# Autodesk Inventor assembly: base_roulante_pmi
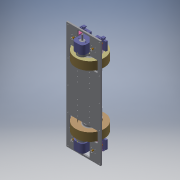
[picture p0: Inventor's stored thumbnail of the model, 180x180]
Saved by Autodesk Inventor 2019 (Build 230136000, 136)
## iProperties
Created: 2020-02-16
Part Number: base_roulante_pmi
Document SubType Name: Assembly
Designer: franc
Author: franc
## Documents named in this file (8)
- C:\Users\franc\Desktop\EsialRobotik\Mecanique\base_roulante\base_roulante_pmi.iam
- C:\Users\franc\Desktop\EsialRobotik\Mecanique\base_roulante\bloc_moteur.iam
- C:\Users\franc\Desktop\EsialRobotik\Mecanique\base_roulante\composants\codeur_S25J.ipt
- C:\Users\franc\Desktop\EsialRobotik\Mecanique\base_roulante\composants\capuchon_roulement.ipt
- C:\Users\franc\Desktop\EsialRobotik\Mecanique\base_roulante\composants\LM4UU.ipt
- C:\Users\franc\Desktop\EsialRobotik\Mecanique\base_roulante\axe_codeur.iam
- C:\Users\franc\Desktop\EsialRobotik\Mecanique\base_roulante\composants\support_codeur S65J.ipt
- C:\Users\franc\Desktop\EsialRobotik\Mecanique\base_roulante\socle_ammovible_pmi.ipt
## Components (19 placed, 7 different names)
1. bloc_moteur:1 [sub-assembly] — Placage:45, Placage:46, Placage:47
2. bloc_moteur:2 [sub-assembly] — Placage:48, Placage:49, Placage:50
3. codeur_S25J:1 — Placage:29, Placage:30, Placage:31
4. capuchon_roulement:1 — Placage:36, Placage:51, Placage:52, Placage:53
5. capuchon_roulement:2 — Placage:54, Placage:55, Placage:56
6. LM4UU:1 — Placage:60, Affleurement:2
7. LM4UU:2 — Placage:61, Affleurement:3
8. LM4UU:3 — Placage:25, Placage:58, Placage:59
9. LM4UU:4 — Placage:26, Placage:57, Affleurement:1
10. axe_codeur:1 [sub-assembly] — Placage:25, Placage:32, Placage:34
11. axe_codeur:2 [sub-assembly] — Placage:26, Placage:33, Placage:35
12. support_codeur S65J:1 — Placage:29, Placage:30, Placage:31, Placage:32, Placage:33, Placage:34, Placage:35, Placage:36
13. socle_ammovible_pmi:1 — Placage:45, Placage:46, Placage:47, Placage:48, Placage:49, Placage:50, Placage:51, Placage:52, Placage:53, Placage:54, Placage:55, Placage:56, Placage:57, Affleurement:1, Placage:58, Placage:59, Placage:60, Affleurement:2, Placage:61, Affleurement:3, Placage:62, Placage:63, Placage:64, Placage:65, Placage:66, Placage:67
14. axe_codeur:3 [sub-assembly] — Placage:71, Placage:73, Placage:75
15. axe_codeur:4 [sub-assembly] — Placage:72, Placage:74, Placage:76
16. capuchon_roulement:3 — Placage:65, Placage:66, Placage:67, Placage:71, Placage:77
17. capuchon_roulement:4 — Placage:62, Placage:63, Placage:64, Placage:72
18. codeur_S25J:2 — Placage:68, Placage:69, Placage:70
19. support_codeur S65J:2 — Placage:68, Placage:69, Placage:70, Placage:73, Placage:74, Placage:75, Placage:76, Placage:77
## Relationships (46: Mate 43, Flush 3)
- Placage:25 [Mate]: LM4UU:3 ↔ axe_codeur:1
- Placage:26 [Mate]: LM4UU:4 ↔ axe_codeur:2
- Placage:29 [Mate]: codeur_S25J:1 ↔ support_codeur S65J:1
- Placage:30 [Mate]: codeur_S25J:1 ↔ support_codeur S65J:1
- Placage:31 [Mate]: codeur_S25J:1 ↔ support_codeur S65J:1
- Placage:32 [Mate]: axe_codeur:1 ↔ support_codeur S65J:1
- Placage:33 [Mate]: axe_codeur:2 ↔ support_codeur S65J:1
- Placage:34 [Mate]: axe_codeur:1 ↔ support_codeur S65J:1
- Placage:35 [Mate]: axe_codeur:2 ↔ support_codeur S65J:1
- Placage:36 [Mate] (8 mm): capuchon_roulement:1 ↔ support_codeur S65J:1
- Placage:45 [Mate]: bloc_moteur:1 ↔ socle_ammovible_pmi:1
- Placage:46 [Mate]: bloc_moteur:1 ↔ socle_ammovible_pmi:1
- Placage:47 [Mate]: bloc_moteur:1 ↔ socle_ammovible_pmi:1
- Placage:48 [Mate]: bloc_moteur:2 ↔ socle_ammovible_pmi:1
- Placage:49 [Mate]: bloc_moteur:2 ↔ socle_ammovible_pmi:1
- Placage:50 [Mate]: bloc_moteur:2 ↔ socle_ammovible_pmi:1
- Placage:51 [Mate]: capuchon_roulement:1 ↔ socle_ammovible_pmi:1
- Placage:52 [Mate]: capuchon_roulement:1 ↔ socle_ammovible_pmi:1
- Placage:53 [Mate]: capuchon_roulement:1 ↔ socle_ammovible_pmi:1
- Placage:54 [Mate]: capuchon_roulement:2 ↔ socle_ammovible_pmi:1
- Placage:55 [Mate]: capuchon_roulement:2 ↔ socle_ammovible_pmi:1
- Placage:56 [Mate]: capuchon_roulement:2 ↔ socle_ammovible_pmi:1
- Placage:57 [Mate]: LM4UU:4 ↔ socle_ammovible_pmi:1
- Affleurement:1 [Flush]: LM4UU:4 ↔ socle_ammovible_pmi:1
- Placage:58 [Mate]: LM4UU:3 ↔ socle_ammovible_pmi:1
- Placage:59 [Mate]: LM4UU:3 ↔ socle_ammovible_pmi:1
- Placage:60 [Mate]: LM4UU:1 ↔ socle_ammovible_pmi:1
- Affleurement:2 [Flush]: LM4UU:1 ↔ socle_ammovible_pmi:1
- Placage:61 [Mate]: LM4UU:2 ↔ socle_ammovible_pmi:1
- Affleurement:3 [Flush]: LM4UU:2 ↔ socle_ammovible_pmi:1
- Placage:62 [Mate]: socle_ammovible_pmi:1 ↔ capuchon_roulement:4
- Placage:63 [Mate]: socle_ammovible_pmi:1 ↔ capuchon_roulement:4
- Placage:64 [Mate]: socle_ammovible_pmi:1 ↔ capuchon_roulement:4
- Placage:65 [Mate]: socle_ammovible_pmi:1 ↔ capuchon_roulement:3
- Placage:66 [Mate]: socle_ammovible_pmi:1 ↔ capuchon_roulement:3
- Placage:67 [Mate]: socle_ammovible_pmi:1 ↔ capuchon_roulement:3
- Placage:68 [Mate]: codeur_S25J:2 ↔ support_codeur S65J:2
- Placage:69 [Mate]: codeur_S25J:2 ↔ support_codeur S65J:2
- Placage:70 [Mate]: codeur_S25J:2 ↔ support_codeur S65J:2
- Placage:71 [Mate]: axe_codeur:3 ↔ capuchon_roulement:3
- Placage:72 [Mate]: axe_codeur:4 ↔ capuchon_roulement:4
- Placage:73 [Mate]: axe_codeur:3 ↔ support_codeur S65J:2
- Placage:74 [Mate]: axe_codeur:4 ↔ support_codeur S65J:2
- Placage:75 [Mate]: axe_codeur:3 ↔ support_codeur S65J:2
- Placage:76 [Mate]: axe_codeur:4 ↔ support_codeur S65J:2
- Placage:77 [Mate] (8 mm): capuchon_roulement:3 ↔ support_codeur S65J:2
